# Autodesk Inventor assembly: Сервопривод с кареткой
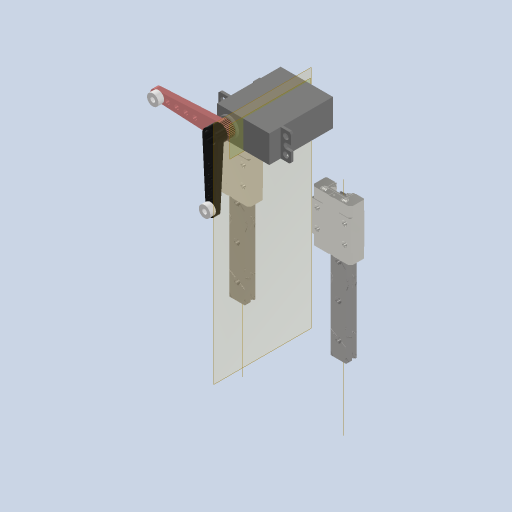
[picture p0: Inventor's stored thumbnail of the model, 512x512]
Saved by Autodesk Inventor 2024.2 (Build 282272000, 272)
## iProperties
Created: 2025-11-27
Part Number: Сервопривод с кареткой
Document SubType Name: Assembly
Designer: katya_notebook
Author: katya_notebook
## Documents named in this file (8)
- C:\Users\91125\OneDrive\Рабочий стол\alletz\3д модель\Сервопривод с кареткой.iam
- C:\Users\91125\OneDrive\Рабочий стол\alletz\3д модель\JX Servo PDI-HV2006MG\JX Servo PDI-HV2006MG.ipt
- C:\Users\91125\OneDrive\Рабочий стол\alletz\3д модель\MGN7C каретка\MGN7C каретка.ipt
- C:\Users\91125\OneDrive\Рабочий стол\alletz\3д модель\MHN7C рельса\MHN7C рельса.ipt
- C:\Users\91125\OneDrive\Рабочий стол\alletz\3д модель\крепление рельс.ipt
- C:\Users\91125\OneDrive\Рабочий стол\alletz\3д модель\крепление каретки.ipt
- C:\Users\91125\OneDrive\Рабочий стол\alletz\3д модель\25T Servo Horn Steering Arm M3.ipt
- C:\Users\91125\OneDrive\Рабочий стол\alletz\3д модель\подшипник мини.ipt
## Components (11 placed, 7 different names)
1. JX Servo PDI-HV2006MG:1 — Совмещение:1, Жесткий:1, Совмещение:5, С поворотом:2
2. MGN7C каретка:1 — Жесткий:2, Совмещение:8
3. MHN7C рельса:1 — Совмещение:2, Заподлицо:1, Совмещение:3, Совмещение:4, Жесткий:2, Совмещение:6, Совмещение:7
4. крепление рельс:1
5. крепление каретки:1
6. 25T Servo Horn Steering Arm M3:1 — Совмещение:1, Жесткий:1, С поворотом:1
7. подшипник мини:1 — С поворотом:1
8. MHN7C рельса:2 — Заподлицо:1, Совмещение:3, Совмещение:6, Совмещение:7, Жесткий:3
9. MGN7C каретка:2 — Жесткий:3, Совмещение:8
10. 25T Servo Horn Steering Arm M3:2 — С поворотом:2, С поворотом:3
11. подшипник мини:2 — С поворотом:3
## Relationships (15: Mate 8, WeldJoint 3, RevoluteJoint 3, Flush 1)
- Совмещение:1 [Mate]: JX Servo PDI-HV2006MG:1 ↔ 25T Servo Horn Steering Arm M3:1
- Жесткий:1 [WeldJoint]: JX Servo PDI-HV2006MG:1 ↔ 25T Servo Horn Steering Arm M3:1
- С поворотом:1 [RevoluteJoint]: 25T Servo Horn Steering Arm M3:1 ↔ подшипник мини:1
- Совмещение:2 [Mate]: MHN7C рельса:1
- Заподлицо:1 [Flush]: MHN7C рельса:1 ↔ MHN7C рельса:2
- Совмещение:3 [Mate] (38 mm): MHN7C рельса:1 ↔ MHN7C рельса:2
- Совмещение:4 [Mate] (22.3 mm): MHN7C рельса:1
- Совмещение:5 [Mate]: JX Servo PDI-HV2006MG:1
- Жесткий:2 [WeldJoint]: MGN7C каретка:1 ↔ MHN7C рельса:1
- Совмещение:6 [Mate]: MHN7C рельса:1 ↔ MHN7C рельса:2
- Совмещение:7 [Mate]: MHN7C рельса:1 ↔ MHN7C рельса:2
- Жесткий:3 [WeldJoint]: MHN7C рельса:2 ↔ MGN7C каретка:2
- Совмещение:8 [Mate]: MGN7C каретка:1 ↔ MGN7C каретка:2
- С поворотом:2 [RevoluteJoint]: JX Servo PDI-HV2006MG:1 ↔ 25T Servo Horn Steering Arm M3:2
- С поворотом:3 [RevoluteJoint]: 25T Servo Horn Steering Arm M3:2 ↔ подшипник мини:2
